# Autodesk Inventor assembly: SideBeam
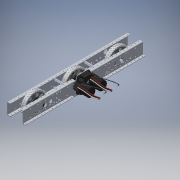
[picture p0: Inventor's stored thumbnail of the model, 180x180]
Saved by Autodesk Inventor 2019 (Build 230136000, 136)
## iProperties
Created: 2020-01-13
Part Number: SideBeam
Document SubType Name: Assembly
Designer: james
Author: james
## Documents named in this file (11)
- F:\JimsRobot\FIRSTRobots\Design\JimsCHS2020FRC\SideBeam.iam
- F:\JimsRobot\FIRSTRobots\Design\Library\AndyMark\am-3922 AM14U4 Inside Plate.ipt
- F:\JimsRobot\FIRSTRobots\Design\Library\AndyMark\Churro 3375.ipt
- F:\JimsRobot\FIRSTRobots\Design\Library\AndyMark\am-3921 AM14U4 Outside Plate.ipt
- F:\JimsRobot\FIRSTRobots\Design\Library\AndyMark\6 HiGrip with bearings, pulleys and spacers.iam
- F:\JimsRobot\FIRSTRobots\Design\Library\AndyMark\6 HiGrip with hub and double pulley.iam
- F:\JimsRobot\FIRSTRobots\Design\Library\AndyMark\FR8ZZ Hex Bearing.ipt
- F:\JimsRobot\FIRSTRobots\Design\Library\AndyMark\FR6ZZ Bearing.ipt
- F:\JimsRobot\FIRSTRobots\Design\Library\AndyMark\TB Output Shaft Hex L-Base 2.ipt
- F:\JimsRobot\FIRSTRobots\Design\Library\AndyMark\TM Housing.ipt
- F:\JimsRobot\FIRSTRobots\Design\Library\RevRobotics\REV-21-1650.ipt
## Components (16 placed, 10 different names)
1. am-3922 AM14U4 Inside Plate:1 — Mate:22, Mate:23, Mate:24, Mate:25, Mate:26, Mate:27, Mate:28, Mate:29, Mate:30, Mate:31, Mate:32, Mate:33, Mate:39, Mate:46, Mate:47, Mate:52
2. Churro 3375:1 — Mate:29, Mate:31, Mate:35
3. Churro 3375:2 — Mate:28, Mate:30
4. Churro 3375:3 — Mate:26, Mate:32, Mate:36
5. Churro 3375:4 — Mate:27, Mate:33
6. am-3921 AM14U4 Outside Plate:1 — Mate:35, Mate:36, Mate:37, Mate:38, Mate:40, Mate:42, Mate:44, Mate:52
7. 6 HiGrip with bearings, pulleys and spacers:1 [sub-assembly] — Mate:42, Mate:44
8. 6 HiGrip with bearings, pulleys and spacers:2 [sub-assembly] — Mate:39, Mate:40
9. 6 HiGrip with hub and double pulley:1 [sub-assembly] — Mate:41, Mate:43
10. FR8ZZ Hex Bearing:1 — Mate:37, Mate:38, Mate:41, Mate:43, Flush:1, Mate:45
11. FR8ZZ Hex Bearing:2 — Mate:22, Mate:23
12. FR6ZZ Bearing:1 — Mate:24, Mate:25
13. TB Output Shaft Hex L-Base 2:1 — Flush:1, Mate:45
14. TM Housing:1 — Mate:46, Mate:47, Mate:48, Mate:49, Mate:50, Mate:51
15. REV-21-1650:1 — Mate:48, Mate:51
16. REV-21-1650:2 — Mate:49, Mate:50
## Relationships (31: Mate 30, Flush 1)
- Mate:22: am-3922 AM14U4 Inside Plate:1 ↔ FR8ZZ Hex Bearing:2
- Mate:23: am-3922 AM14U4 Inside Plate:1 ↔ FR8ZZ Hex Bearing:2
- Mate:24: am-3922 AM14U4 Inside Plate:1 ↔ FR6ZZ Bearing:1
- Mate:25: am-3922 AM14U4 Inside Plate:1 ↔ FR6ZZ Bearing:1
- Mate:26: am-3922 AM14U4 Inside Plate:1 ↔ Churro 3375:3
- Mate:27: am-3922 AM14U4 Inside Plate:1 ↔ Churro 3375:4
- Mate:28: am-3922 AM14U4 Inside Plate:1 ↔ Churro 3375:2
- Mate:29: am-3922 AM14U4 Inside Plate:1 ↔ Churro 3375:1
- Mate:30: am-3922 AM14U4 Inside Plate:1 ↔ Churro 3375:2
- Mate:31: am-3922 AM14U4 Inside Plate:1 ↔ Churro 3375:1
- Mate:32: am-3922 AM14U4 Inside Plate:1 ↔ Churro 3375:3
- Mate:33: am-3922 AM14U4 Inside Plate:1 ↔ Churro 3375:4
- Mate:35: Churro 3375:1 ↔ am-3921 AM14U4 Outside Plate:1
- Mate:36: Churro 3375:3 ↔ am-3921 AM14U4 Outside Plate:1
- Mate:37: am-3921 AM14U4 Outside Plate:1 ↔ FR8ZZ Hex Bearing:1
- Mate:38: am-3921 AM14U4 Outside Plate:1 ↔ FR8ZZ Hex Bearing:1
- Mate:39: am-3922 AM14U4 Inside Plate:1 ↔ 6 HiGrip with bearings, pulleys and spacers:2
- Mate:40: am-3921 AM14U4 Outside Plate:1 ↔ 6 HiGrip with bearings, pulleys and spacers:2
- Mate:41: 6 HiGrip with hub and double pulley:1 ↔ FR8ZZ Hex Bearing:1
- Mate:42: am-3921 AM14U4 Outside Plate:1 ↔ 6 HiGrip with bearings, pulleys and spacers:1
- Mate:43: 6 HiGrip with hub and double pulley:1 ↔ FR8ZZ Hex Bearing:1
- Mate:44: am-3921 AM14U4 Outside Plate:1 ↔ 6 HiGrip with bearings, pulleys and spacers:1
- Flush:1: FR8ZZ Hex Bearing:1 ↔ TB Output Shaft Hex L-Base 2:1
- Mate:45: FR8ZZ Hex Bearing:1 ↔ TB Output Shaft Hex L-Base 2:1
- Mate:46: am-3922 AM14U4 Inside Plate:1 ↔ TM Housing:1
- Mate:47: am-3922 AM14U4 Inside Plate:1 ↔ TM Housing:1
- Mate:48: TM Housing:1 ↔ REV-21-1650:1
- Mate:49: TM Housing:1 ↔ REV-21-1650:2
- Mate:50: TM Housing:1 ↔ REV-21-1650:2
- Mate:51: TM Housing:1 ↔ REV-21-1650:1
- Mate:52 (76.2 mm): am-3922 AM14U4 Inside Plate:1 ↔ am-3921 AM14U4 Outside Plate:1
